# Autodesk Inventor assembly: FullElevator
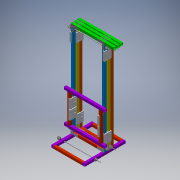
[picture p0: Inventor's stored thumbnail of the model, 180x180]
Saved by Autodesk Inventor 2019 (Build 230136000, 136)
## iProperties
Created: 2019-01-09
Part Number: FullElevator
Document SubType Name: Assembly
Designer: james
Mass: 6156.31 g
Surface Area: 24705.8 cm^2
Volume: 2575.87 cm^3
Density: 2.38999 g/cm^3
Author: james
## Documents named in this file (6)
- F:\JimsDesign\2019CHS4089\FullElevator.iam
- F:\JimsDesign\2019CHS4089\ElvMiddleFrame.iam
- F:\JimsDesign\2019CHS4089\ElvFixedFrame.iam
- F:\JimsDesign\2019CHS4089\BaseFrame.iam
- F:\JimsDesign\2019CHS4089\ElvFrontFrame.iam
- F:\JimsDesign\2019CHS4089\ElvEndEffectFrame.iam
## Components (5 placed, 5 different names)
1. ElvMiddleFrame:1 [sub-assembly] — Mate:1, Mate:2, Mate:3, Flush:1
2. ElvFixedFrame:1 [sub-assembly] — Mate:1, Mate:2
3. BaseFrame:1 [sub-assembly]
4. ElvFrontFrame:1 [sub-assembly] — Mate:3, Flush:1, Mate:4, Flush:2
5. ElvEndEffectFrame:1 [sub-assembly] — Mate:4, Flush:2
## Relationships (6: Mate 4, Flush 2)
- Mate:1: ElvMiddleFrame:1 ↔ ElvFixedFrame:1
- Mate:2 (8.89 mm): ElvMiddleFrame:1 ↔ ElvFixedFrame:1
- Mate:3 (12.7 mm): ElvMiddleFrame:1 ↔ ElvFrontFrame:1
- Flush:1: ElvMiddleFrame:1 ↔ ElvFrontFrame:1
- Mate:4 (10.16 mm): ElvFrontFrame:1 ↔ ElvEndEffectFrame:1
- Flush:2: ElvFrontFrame:1 ↔ ElvEndEffectFrame:1
